# Autodesk Inventor assembly: ASM_Micron_Rev2(manipulator)
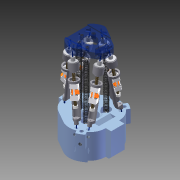
[picture p0: Inventor's stored thumbnail of the model, 180x180]
Saved by Autodesk Inventor 2011 SP2 (Build 150309200, 309)
## iProperties
Created: 2012-01-18
Part Number: ASM_Micron_Rev2(manipulator)
Document SubType Name: Assembly
Designer: sungwook
Author: sungwook
## Documents named in this file (8)
- C:\Users\sungwook\Documents\Inventor\Micron22_top_adj_02082013\Assembly\ASM_Micron_Rev2(manipulator).iam
- C:\Users\sungwook\Documents\Inventor\Micron22_top_adj_02082013\Parts\Main\Platform_Base_20mm_Rev2.ipt
- C:\Users\sungwook\Documents\Inventor\Micron22_top_adj_02082013\Parts\Main\Platform_Top_14mm_Rev.ipt
- C:\Users\sungwook\Documents\Inventor\Micron22_top_adj_02082013\Parts\Tool\ASM_Tool_Tip_Rev.iam
- C:\Users\sungwook\Documents\Inventor\Micron22_top_adj_02082013\Assembly\ASM_Motor_Unit_Rev.iam
- C:\Users\sungwook\Documents\Inventor\Micron22_top_adj_02082013\Parts\Main\Eye_Pin_26Ga.ipt
- C:\Users\sungwook\Documents\Inventor\Content Center Files\R2011\en-US\ANSI B18.6.3(12)\ANSI B18.6.3 - 0-80 UNF - 0.1875(15_).ipt
- C:\Users\sungwook\Documents\Inventor\Micron22_top_adj_02082013\Parts\Main\Spring.ipt
## Components (21 placed, 7 different names)
1. Platform_Base_20mm_Rev2:1 — Mate:4, Mate:6, Mate:8, Angle:1, Mate:14, Flush:15
2. Platform_Top_14mm_Rev:1 — Mate:1, Mate:2, Mate:3, Mate:4, Mate:5, Mate:7, Angle:1, Mate:9, Mate:10, Angle:2
3. ASM_Tool_Tip_Rev:1 [sub-assembly] — Mate:1, Mate:2, Mate:3, Mate:11
4. ASM_Motor_Unit_Rev:1 [sub-assembly] — Mate:5, Mate:6
5. ASM_Motor_Unit_Rev:2 [sub-assembly] — Mate:7, Mate:8
6. ASM_Motor_Unit_Rev:3 [sub-assembly]
7. ASM_Motor_Unit_Rev:4 [sub-assembly]
8. ASM_Motor_Unit_Rev:5 [sub-assembly]
9. ASM_Motor_Unit_Rev:6 [sub-assembly]
10. Cross Recessed Flat Countersunk Head Machine Screw - Type I - Inch 0-80 x 3/16:1 — Mate:11
11. Cross Recessed Flat Countersunk Head Machine Screw - Type I - Inch 0-80 x 3/16:2
12. Cross Recessed Flat Countersunk Head Machine Screw - Type I - Inch 0-80 x 3/16:3
13. Eye_Pin_26Ga:1 — Mate:9, Mate:10, Angle:2, Mate:12, Mate:15
14. Spring:1 — Mate:12, Mate:15
15. Eye_Pin_26Ga:4 — Mate:14, Flush:15
16. Eye_Pin_26Ga:5
17. Spring:2
18. Eye_Pin_26Ga:6
19. Eye_Pin_26Ga:7
20. Spring:3
21. Eye_Pin_26Ga:8
## Component patterns: (3 elements, first: ASM_Motor_Unit_Rev:1 + ASM_Motor_Unit_Rev:2), Tool Mount Bolts (3 elements), (3 elements, first: Eye_Pin_26Ga:1 + Spring:1 + Eye_Pin_26Ga:4)
## Relationships (17: Mate 14, Angle 2, Flush 1)
- Mate:1: Platform_Top_14mm_Rev:1 ↔ ASM_Tool_Tip_Rev:1
- Mate:2: Platform_Top_14mm_Rev:1 ↔ ASM_Tool_Tip_Rev:1
- Mate:3: Platform_Top_14mm_Rev:1 ↔ ASM_Tool_Tip_Rev:1
- Mate:4: Platform_Base_20mm_Rev2:1 ↔ Platform_Top_14mm_Rev:1
- Mate:5: Platform_Top_14mm_Rev:1 ↔ ASM_Motor_Unit_Rev:1
- Mate:6: Platform_Base_20mm_Rev2:1 ↔ ASM_Motor_Unit_Rev:1
- Mate:7: Platform_Top_14mm_Rev:1 ↔ ASM_Motor_Unit_Rev:2
- Mate:8: Platform_Base_20mm_Rev2:1 ↔ ASM_Motor_Unit_Rev:2
- Angle:1 (180 deg): Platform_Base_20mm_Rev2:1 ↔ Platform_Top_14mm_Rev:1
- Mate:9: Platform_Top_14mm_Rev:1 ↔ Eye_Pin_26Ga:1
- Mate:10: Platform_Top_14mm_Rev:1 ↔ Eye_Pin_26Ga:1
- Angle:2 (0 deg): Platform_Top_14mm_Rev:1 ↔ Eye_Pin_26Ga:1
- Mate:12: Eye_Pin_26Ga:1 ↔ Spring:1
- Mate:14: Platform_Base_20mm_Rev2:1 ↔ Eye_Pin_26Ga:4
- Flush:15: Platform_Base_20mm_Rev2:1 ↔ Eye_Pin_26Ga:4
- Mate:15: Eye_Pin_26Ga:1 ↔ Spring:1
- Mate:11: ASM_Tool_Tip_Rev:1 ↔ Cross Recessed Flat Countersunk Head Machine Screw - Type I - Inch 0-80 x 3/16:1
